# Autodesk Inventor assembly: GE-12017
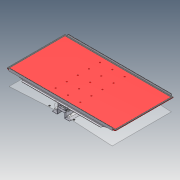
[picture p0: Inventor's stored thumbnail of the model, 180x180]
Saved by Autodesk Inventor 2012 (Build 160160000, 160)
## iProperties
Created: 2011-06-06
Part Number: GE-12017
Document SubType Name: Assembly
Designer: dfoster
Description: Bridge Assembly
Title: Bridge Assembly
Author: dfoster
## Documents named in this file (11)
- C:\Data Folder\FRC 2012 Field\Components\GE-12017.iam
- C:\Data Folder\FRC 2012 Field\Components\GE-12018.ipt
- C:\Data Folder\FRC 2012 Field\Components\GE-12022.iam
- C:\Data Folder\FRC 2012 Field\Components\GE-12019.iam
- C:\Data Folder\FRC 2012 Field\Components\GE-12095.ipt
- C:\Data Folder\FRC 2012 Field\Components\GE-12017-01.ipt
- C:\Data Folder\FRC 2012 Field\Components\GE-12017-02.ipt
- C:\Data Folder\FRC 2012 Field\Components\HW-00072.ipt
- C:\Data Folder\FRC 2012 Field\Components\HW-00026.ipt
- C:\Data Folder\FRC 2012 Field\Components\GE-12017-03.ipt
- C:\Data Folder\FRC 2012 Field\Components\GE-12064.iam
## Components (13 placed, 10 different names)
1. GE-12018:1 — Mate:2, Flush:3, Flush:5, Flush:6, Flush:8, Mate:6, Flush:9, Flush:10
2. GE-12095:1 — Flush:5, Flush:6, Mate:7, Flush:11, Flush:12
3. GE-12017-01:1 — Mate:6, Flush:9, Flush:10, Mate:8
4. GE-12017-02:1 — Mate:7, Flush:11, Flush:12, Mate:8
5. GE-12022:1 [sub-assembly] — Mate:3, Mate:4, Flush:2, Mate:5, Flush:3, Insert:1, Insert:2, Insert:3, Insert:4, Mate:11, Mate:12, Mate:13, Mate:14, Mate:15, Mate:16
6. GE-12019:1 [sub-assembly] — Mate:2, Mate:3, Mate:4, Flush:2, Flush:7, Mate:9, Flush:13, Flush:14, Flush:15, Flush:16
7. HW-00072:1 — Insert:1
8. HW-00072:2 — Insert:2
9. HW-00026:1 — Insert:4
10. HW-00026:2 — Insert:3
11. GE-12017-03:1 — Mate:9, Flush:13, Flush:14
12. GE-12064:1 [sub-assembly] — Mate:11, Mate:12, Mate:13, Flush:15
13. GE-12064:2 [sub-assembly] — Flush:16, Mate:14, Mate:15, Mate:16
## Relationships (33: Mate 15, Flush 14, Insert 4)
- [Mate]: GE-12018:1 ↔ GE-12019:1
- Mate:2 (6.35 mm): GE-12018:1 ↔ GE-12019:1
- Mate:3: GE-12022:1 ↔ GE-12019:1
- Mate:4: GE-12022:1 ↔ GE-12019:1
- Flush:2: GE-12022:1 ↔ GE-12019:1
- Mate:5: GE-12022:1
- Flush:3 (-1041.4 mm): GE-12018:1 ↔ GE-12022:1
- Flush:5: GE-12018:1 ↔ GE-12095:1
- Flush:6: GE-12018:1 ↔ GE-12095:1
- Flush:7 (-609.6 mm): GE-12019:1
- Flush:8 (1117.6 mm): GE-12018:1
- Mate:6: GE-12018:1 ↔ GE-12017-01:1
- Flush:9: GE-12018:1 ↔ GE-12017-01:1
- Flush:10: GE-12018:1 ↔ GE-12017-01:1
- Mate:7: GE-12095:1 ↔ GE-12017-02:1
- Flush:11: GE-12095:1 ↔ GE-12017-02:1
- Flush:12: GE-12095:1 ↔ GE-12017-02:1
- Mate:8: GE-12017-01:1 ↔ GE-12017-02:1
- Insert:1: GE-12022:1 ↔ HW-00072:1
- Insert:2: GE-12022:1 ↔ HW-00072:2
- Insert:3: GE-12022:1 ↔ HW-00026:2
- Insert:4: GE-12022:1 ↔ HW-00026:1
- Mate:9 (-0.7937 mm): GE-12019:1 ↔ GE-12017-03:1
- Flush:13 (12.7 mm): GE-12019:1 ↔ GE-12017-03:1
- Flush:14: GE-12019:1 ↔ GE-12017-03:1
- Mate:11 (12.7 mm): GE-12022:1 ↔ GE-12064:1
- Mate:12: GE-12022:1 ↔ GE-12064:1
- Mate:13: GE-12022:1 ↔ GE-12064:1
- Flush:15: GE-12019:1 ↔ GE-12064:1
- Flush:16: GE-12019:1 ↔ GE-12064:2
- Mate:14 (12.7 mm): GE-12022:1 ↔ GE-12064:2
- Mate:15: GE-12022:1 ↔ GE-12064:2
- Mate:16: GE-12022:1 ↔ GE-12064:2
